# Autodesk Inventor assembly: Baugruppe_Zerstäuber
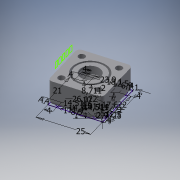
[picture p0: Inventor's stored thumbnail of the model, 180x180]
Saved by Autodesk Inventor 2019 (Build 230136000, 136)
## iProperties
Created: 2018-09-03
Part Number: Baugruppe_Zerstäuber
Material: Generisch
Document SubType Name: Assembly
Designer: kenoe
Author: kenoe
## Documents named in this file (9)
- C:\Users\kenoe\OneDrive\Dokumente\Baugruppe_Zerstäuber.iam
- C:\Users\kenoe\OneDrive\Dokumente\Unterteil_Zerstäuber.ipt
- C:\Users\kenoe\OneDrive\Dokumente\Oberteil_Zerstäuber_MIR.ipt
- C:\Users\kenoe\OneDrive\Dokumente\Fitting_Zerstäuber.ipt
- C:\Users\kenoe\OneDrive\Dokumente\Zerstäuber_Luer_Lock.ipt
- C:\Users\kenoe\OneDrive\Dokumente\Baugruppe_Zerstäuber\Konstruktions-Assistent\Schraubenverbindung7.iam
- C:\Users\kenoe\OneDrive\Dokumente\Baugruppe_Zerstäuber\Konstruktions-Assistent\Schraubenverbindung8.iam
- C:\Users\kenoe\OneDrive\Dokumente\Baugruppe_Zerstäuber\Konstruktions-Assistent\Schraubenverbindung9.iam
- C:\Users\kenoe\OneDrive\Dokumente\Baugruppe_Zerstäuber\Konstruktions-Assistent\Schraubenverbindung10.iam
## Components (8 placed, 5 different names)
1. Unterteil_Zerstäuber:1 — Einfügen:1, Einfügen:4, Passend:4, Passend:6, Passend:8, Passend:10
2. Oberteil_Zerstäuber_MIR:1 — Einfügen:1, Winkel:1, Tangential:1, Einfügen:2, Einfügen:3, Einfügen:4, Passend:3, Passend:5, Passend:7, Passend:9
3. Fitting_Zerstäuber:1 — Fluchtend:1, Einfügen:2
4. Zerstäuber_Luer_Lock:1 — Einfügen:3
5. Schraubenverbindung:2 [sub-assembly] — Passend:3, Passend:4
6. Schraubenverbindung:3 [sub-assembly] — Passend:5, Passend:6
7. Schraubenverbindung:4 [sub-assembly] — Passend:7, Passend:8
8. Schraubenverbindung:5 [sub-assembly] — Passend:9, Passend:10
## Relationships (15: Mate 8, Insert 4, Flush 1, Angle 1, Tangent 1)
- Einfügen:1 [Insert]: Unterteil_Zerstäuber:1 ↔ Oberteil_Zerstäuber_MIR:1
- Fluchtend:1 [Flush] (5.719 mm): Fitting_Zerstäuber:1
- Winkel:1 [Angle] (0 deg): Oberteil_Zerstäuber_MIR:1
- Tangential:1: Oberteil_Zerstäuber_MIR:1
- Einfügen:2 [Insert] (-2.442 mm): Oberteil_Zerstäuber_MIR:1 ↔ Fitting_Zerstäuber:1
- Einfügen:3 [Insert]: Oberteil_Zerstäuber_MIR:1 ↔ Zerstäuber_Luer_Lock:1
- Einfügen:4 [Insert] (-8 mm): Unterteil_Zerstäuber:1 ↔ Oberteil_Zerstäuber_MIR:1
- Passend:3 [Mate]: Oberteil_Zerstäuber_MIR:1 ↔ Schraubenverbindung:2
- Passend:4 [Mate]: Unterteil_Zerstäuber:1 ↔ Schraubenverbindung:2
- Passend:5 [Mate]: Oberteil_Zerstäuber_MIR:1 ↔ Schraubenverbindung:3
- Passend:6 [Mate]: Unterteil_Zerstäuber:1 ↔ Schraubenverbindung:3
- Passend:7 [Mate]: Oberteil_Zerstäuber_MIR:1 ↔ Schraubenverbindung:4
- Passend:8 [Mate]: Unterteil_Zerstäuber:1 ↔ Schraubenverbindung:4
- Passend:9 [Mate]: Oberteil_Zerstäuber_MIR:1 ↔ Schraubenverbindung:5
- Passend:10 [Mate]: Unterteil_Zerstäuber:1 ↔ Schraubenverbindung:5
